# Autodesk Inventor assembly: BBP
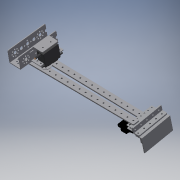
[picture p0: Inventor's stored thumbnail of the model, 180x180]
Saved by Autodesk Inventor 2016 (Build 200138000, 138)
## iProperties
Created: 2016-09-30
Part Number: BBP
Document SubType Name: Assembly
Designer: Delta
Author: Delta
## Documents named in this file (10)
- C:\Robotics\CAD\2016-17_CAD\BBP.iam
- C:\Robotics\CAD\COTSParts\Tetrix\Tetrix channel 160mm.ipt
- C:\Robotics\CAD\COTSParts\Tetrix\Tetrix flat bar 288mm.ipt
- C:\Robotics\CAD\COTSParts\Tetrix\Tetrix bracket - single servo.ipt
- C:\Robotics\CAD\COTSParts\Actobotics\585 parts\585382.ipt
- C:\Robotics\CAD\COTSParts\Tetrix\Tetrix servo 180.ipt
- C:\Robotics\CAD\2015-16_CAD\Part5.ipt
- C:\Robotics\CAD\2015-16_CAD\Part6.ipt
- C:\Robotics\CAD\2015-16_CAD\Tetrix angle 144mm_3in.ipt
- C:\Robotics\CAD\COTSParts\ModernRobotics\45-2006_ODS.ipt
## Components (11 placed, 9 different names)
1. Tetrix channel 160mm:2 — Insert:11, Insert:14, Insert:16, Insert:17
2. Tetrix flat bar 288mm:1 — Insert:12, Insert:13
3. Tetrix flat bar 288mm:2 — Insert:10, Mate:5
4. Tetrix bracket - single servo:1 — Mate:1, Flush:1, Flush:2, Insert:14, Insert:16
5. Tetrix servo 180:1 — Mate:1, Flush:1, Flush:2, Mate:5
6. 585382:5 — Insert:9, Insert:10, Insert:13, Mate:4, Insert:15
7. Part5:1 — Insert:11, Insert:12, Insert:17
8. Part6:1 — Mate:2, Flush:5, Flush:6
9. Tetrix angle 144mm_3in:1 — Insert:9, Flush:7, Flush:8, Mate:3
10. Tetrix angle 144mm_3in:2 — Mate:2, Flush:5, Flush:6, Flush:7, Flush:8, Mate:3
11. 45-2006_ODS:1 — Mate:4, Insert:15
## Relationships (20: Insert 9, Flush 6, Mate 5)
- Mate:1 (5.3594 mm): Tetrix bracket - single servo:1 ↔ Tetrix servo 180:1
- Flush:1: Tetrix bracket - single servo:1 ↔ Tetrix servo 180:1
- Flush:2: Tetrix bracket - single servo:1 ↔ Tetrix servo 180:1
- Mate:2: Part6:1 ↔ Tetrix angle 144mm_3in:2
- Flush:5: Part6:1 ↔ Tetrix angle 144mm_3in:2
- Flush:6: Part6:1 ↔ Tetrix angle 144mm_3in:2
- Insert:9: 585382:5 ↔ Tetrix angle 144mm_3in:1
- Flush:7: Tetrix angle 144mm_3in:1 ↔ Tetrix angle 144mm_3in:2
- Flush:8: Tetrix angle 144mm_3in:1 ↔ Tetrix angle 144mm_3in:2
- Mate:3: Tetrix angle 144mm_3in:1 ↔ Tetrix angle 144mm_3in:2
- Insert:10: Tetrix flat bar 288mm:2 ↔ 585382:5
- Insert:11: Tetrix channel 160mm:2 ↔ Part5:1
- Insert:12: Tetrix flat bar 288mm:1 ↔ Part5:1
- Insert:13: Tetrix flat bar 288mm:1 ↔ 585382:5
- Insert:14: Tetrix channel 160mm:2 ↔ Tetrix bracket - single servo:1
- Mate:4: 585382:5 ↔ 45-2006_ODS:1
- Insert:15: 585382:5 ↔ 45-2006_ODS:1
- Insert:16: Tetrix channel 160mm:2 ↔ Tetrix bracket - single servo:1
- Insert:17: Tetrix channel 160mm:2 ↔ Part5:1
- Mate:5: Tetrix flat bar 288mm:2 ↔ Tetrix servo 180:1
